# Autodesk Inventor assembly: First_Floor
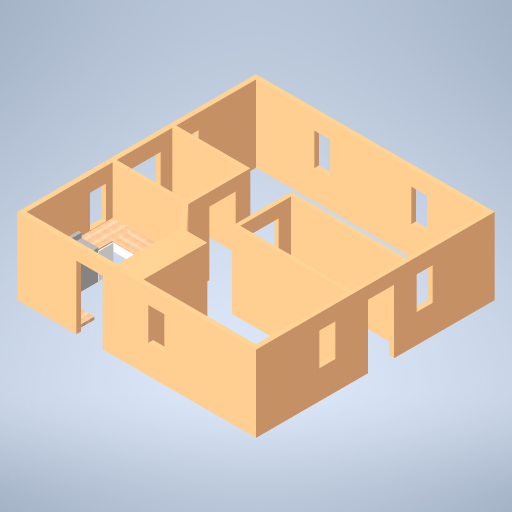
[picture p0: Inventor's stored thumbnail of the model, 512x512]
Saved by Autodesk Inventor 2024 (Build 280153000, 153)
## iProperties
Created: 2023-05-06
Part Number: First_Floor
Document SubType Name: Assembly
Designer: Tom
Author: Tom
## Documents named in this file (7)
- C:\Users\Tom\Documents\Tom_Levers_Public_Git_Repository\Inventor\Mobility\First_Floor.iam
- C:\Users\Tom\Documents\Tom_Levers_Public_Git_Repository\Inventor\Mobility\Walls--First_Floor.ipt
- C:\Users\Tom\Documents\Tom_Levers_Public_Git_Repository\Inventor\Mobility\Stand--Sink_and_Corner_Cabinets.ipt
- C:\Users\Tom\Documents\Tom_Levers_Public_Git_Repository\Inventor\Mobility\Corner_Cabinet.ipt
- C:\Users\Tom\Documents\Tom_Levers_Public_Git_Repository\Inventor\Mobility\Window_Cabinet\Window_Cabinet.iam
- C:\Users\Tom\Documents\Tom_Levers_Public_Git_Repository\Inventor\Mobility\Dishwasher.ipt
- C:\Users\Tom\Documents\Tom_Levers_Public_Git_Repository\Inventor\Mobility\Range.ipt
## Components (6 placed, 6 different names)
1. Walls--First_Floor:1 — Flush:1, Flush:3, Mate:12, Mate:13, Mate:14, Mate:15, Mate:16, Mate:17, Mate:21, Flush:4, Flush:5
2. Stand--Sink_and_Corner_Cabinets:1 — Flush:1, Mate:5, Mate:14, Mate:15
3. Corner_Cabinet:1 — Mate:5, Mate:12, Mate:13, Mate:22
4. Window_Cabinet:1 [sub-assembly] — Flush:3, Mate:16, Mate:17, Mate:18, Mate:20
5. Dishwasher:1 — Mate:18, Mate:20, Flush:5
6. Range:1 — Mate:21, Mate:22, Flush:4
## Relationships (15: Mate 11, Flush 4)
- Flush:1: Walls--First_Floor:1 ↔ Stand--Sink_and_Corner_Cabinets:1
- Mate:5: Stand--Sink_and_Corner_Cabinets:1 ↔ Corner_Cabinet:1
- Flush:3: Walls--First_Floor:1 ↔ Window_Cabinet:1
- Mate:12: Walls--First_Floor:1 ↔ Corner_Cabinet:1
- Mate:13: Walls--First_Floor:1 ↔ Corner_Cabinet:1
- Mate:14: Walls--First_Floor:1 ↔ Stand--Sink_and_Corner_Cabinets:1
- Mate:15: Walls--First_Floor:1 ↔ Stand--Sink_and_Corner_Cabinets:1
- Mate:16: Walls--First_Floor:1 ↔ Window_Cabinet:1
- Mate:17: Walls--First_Floor:1 ↔ Window_Cabinet:1
- Mate:18: Window_Cabinet:1 ↔ Dishwasher:1
- Mate:20: Window_Cabinet:1 ↔ Dishwasher:1
- Mate:21: Walls--First_Floor:1 ↔ Range:1
- Mate:22 (3.175 mm): Corner_Cabinet:1 ↔ Range:1
- Flush:4: Walls--First_Floor:1 ↔ Range:1
- Flush:5: Walls--First_Floor:1 ↔ Dishwasher:1
